# Autodesk Inventor assembly: PTO_PistonMech
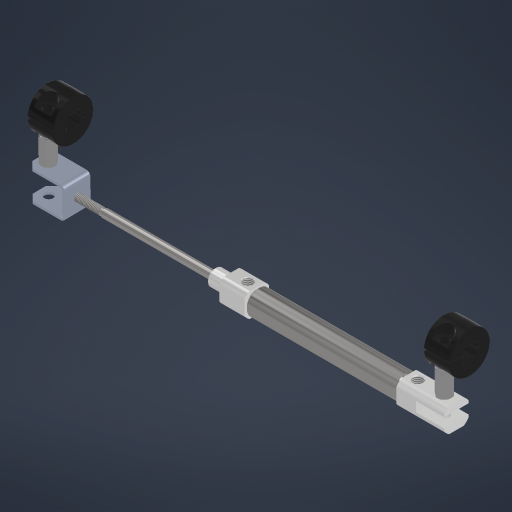
[picture p0: Inventor's stored thumbnail of the model, 512x512]
Saved by Autodesk Inventor 2023.4 (Build 274418000, 418)
## iProperties
Created: 2024-03-13
Part Number: PTO_PistonMech
Document SubType Name: Assembly
Designer: Meer
Author: Meer
## Documents named in this file (6)
- C:\Users\Meer\OneDrive\Documents\GitHub\2024-599Z\Cad\worlds bot possibly\Drivebase\Assembly\Sub-Assembly\PTO_PistonMech.iam
- C:\Users\Meer\OneDrive\Documents\GitHub\2024-599Z\Cad\Library\VEX-CAD-Inventor-1.4.0\Structure\Standoff\Standoff .50.ipt
- C:\Users\Meer\OneDrive\Documents\GitHub\2024-599Z\Cad\Library\VEX-CAD-Inventor-1.4.0\Structure\Standoff.ipt
- C:\Users\Meer\OneDrive\Documents\GitHub\2024-599Z\Cad\Library\VEX-CAD-Inventor-1.4.0\Motion\Pneumatics\Cylinder Mount.ipt
- C:\Users\Meer\OneDrive\Documents\GitHub\2024-599Z\Cad\Library\VEX-CAD-Inventor-1.4.0\Motion\Shaft HS\HS Shaft Collar.ipt
- C:\Users\Meer\OneDrive\Documents\GitHub\2024-599Z\Cad\Library\VEX-CAD-Inventor-1.4.0\Motion\Pneumatics\Double Acting Piston.iam
## Components (6 placed, 4 different names)
1. Standoff .50:1 — Insert:2, Insert:3
2. Cylinder Mount:1 — Insert:1, Insert:2
3. HS Shaft Collar:1 — Insert:3
4. Standoff .50:2 — Insert:4, Insert:5
5. Double Acting Piston:2 [sub-assembly] — Insert:1, Insert:4
6. HS Shaft Collar:3 — Insert:5
## Relationships (5: Insert 5)
- Insert:1 (-2.921 mm): Cylinder Mount:1 ↔ Double Acting Piston:2
- Insert:2: Standoff .50:1 ↔ Cylinder Mount:1
- Insert:3: Standoff .50:1 ↔ HS Shaft Collar:1
- Insert:4: Standoff .50:2 ↔ Double Acting Piston:2
- Insert:5: Standoff .50:2 ↔ HS Shaft Collar:3
